# Autodesk Inventor assembly: strain sensor with lm and wires
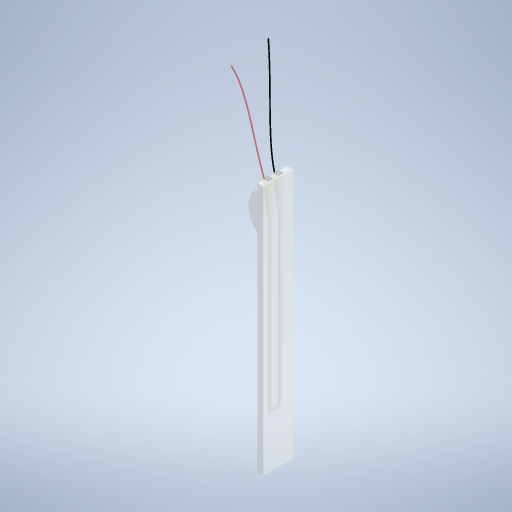
[picture p0: Inventor's stored thumbnail of the model, 512x512]
Saved by Autodesk Inventor 2024.2 (Build 282272000, 272)
## iProperties
Created: 2025-02-11
Part Number: strain sensor with lm and wires
Document SubType Name: Assembly
Designer: Tom
Author: Tom
## Documents named in this file (4)
- C:\Users\Tom\Desktop\UCSF\Preeya UCB\stretchable project\Strain-Sensor-\CAD Files\sensor fab\strain sensor with lm and wires.iam
- C:\Users\Tom\Desktop\UCSF\Preeya UCB\stretchable project\Strain-Sensor-\CAD Files\sensor fab\strain sensor silicone.ipt
- C:\Users\Tom\Desktop\UCSF\Preeya UCB\stretchable project\Strain-Sensor-\CAD Files\sensor fab\basic strain gauge 0p02.ipt
- C:\Users\Tom\Desktop\UCSF\Preeya UCB\stretchable project\Strain-Sensor-\CAD Files\sensor fab\wire.ipt
## Components (4 placed, 3 different names)
1. strain sensor silicone:1 — Flush:1, Flush:2, Mate:1
2. basic strain gauge 0p02:1 — Flush:1, Flush:2, Mate:1, Mate:2, Mate:3
3. wire:1 — Mate:2
4. wire:2 — Mate:3
## Relationships (5: Mate 3, Flush 2)
- Flush:1 (0.508 mm): strain sensor silicone:1 ↔ basic strain gauge 0p02:1
- Flush:2 (2.159 mm): strain sensor silicone:1 ↔ basic strain gauge 0p02:1
- Mate:1: strain sensor silicone:1 ↔ basic strain gauge 0p02:1
- Mate:2 (-2.54 mm): basic strain gauge 0p02:1 ↔ wire:1
- Mate:3 (-2.54 mm): basic strain gauge 0p02:1 ↔ wire:2
